# Autodesk Inventor assembly: SUBFrameBottom
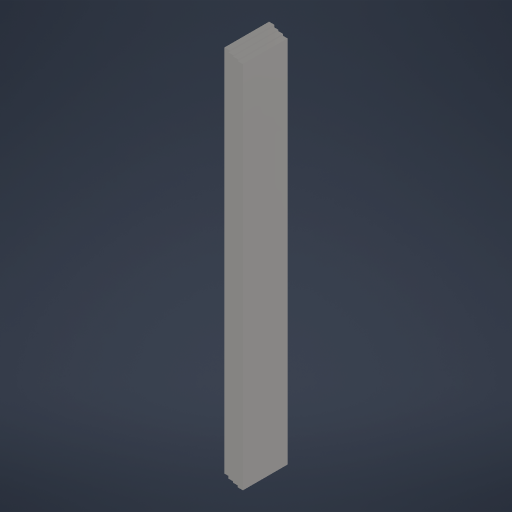
[picture p0: Inventor's stored thumbnail of the model, 512x512]
Saved by Autodesk Inventor 2024 (Build 280153000, 153)
## iProperties
Created: 2025-02-07
Part Number: SUBFrameBottom
Document SubType Name: Assembly
Designer: Tommy Rohmann
Author: Tommy Rohmann
## Documents named in this file (3)
- C:\Users\Tommy Rohmann\OneDrive\Projects\Microgravity-Press-Washing-Machine\System Design and Documentation\Inventor Design Project\SUBFrameBottom.iam
- C:\Users\Tommy Rohmann\OneDrive\Projects\Microgravity-Press-Washing-Machine\System Design and Documentation\Inventor Design Project\LAYOUT.ipt
- C:\Users\Tommy Rohmann\OneDrive\Projects\Microgravity-Press-Washing-Machine\System Design and Documentation\Inventor Design Project\FrameBottomBeam.ipt
## Components (5 placed, 2 different names)
1. LAYOUT:1
2. FrameBottomBeam:1 — Mate:1
3. FrameBottomBeam:2 — Mate:3
4. FrameBottomBeam:3 — Mate:2, Mate:3
5. FrameBottomBeam:4 — Mate:1, Mate:2
## Relationships (4: Mate 3, Composite 1)
- [Composite]: LAYOUT:1 ↔ FrameBottomBeam:1
- Mate:1: FrameBottomBeam:1 ↔ FrameBottomBeam:4
- Mate:2: FrameBottomBeam:3 ↔ FrameBottomBeam:4
- Mate:3: FrameBottomBeam:2 ↔ FrameBottomBeam:3
